# Autodesk Inventor assembly: Frame
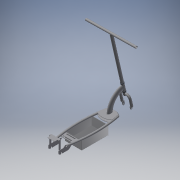
[picture p0: Inventor's stored thumbnail of the model, 180x180]
Saved by Autodesk Inventor 2018 (Build 220112000, 112)
## iProperties
Created: 2018-08-10
Part Number: Frame
Document SubType Name: Assembly
Designer: ruben
Author: ruben
## Documents named in this file (11)
- C:\Users\ruben\Documents\Inventor\Electric-Scooter\Frame\Frame.iam
- C:\Users\ruben\Documents\Inventor\Electric-Scooter\Frame\Rear Wheel Holder.ipt
- C:\Users\ruben\Documents\Inventor\Electric-Scooter\Frame\Footboard - feet protect holder.ipt
- C:\Users\ruben\Documents\Inventor\Electric-Scooter\Frame\Batterybox 2\Batterybox 2.ipt
- C:\Users\ruben\Documents\Inventor\Electric-Scooter\Frame\Tubes.ipt
- C:\Users\ruben\Documents\Inventor\Electric-Scooter\Frame\Handle bars\Handle bars holder plates.ipt
- C:\Users\ruben\Documents\Inventor\Electric-Scooter\Frame\Handle bars\Handle bars holder.ipt
- C:\Users\ruben\Documents\Inventor\Electric-Scooter\Frame\Handle bars\Handle bars holder axle.ipt
- C:\Users\ruben\Documents\Inventor\Electric-Scooter\Transmission\Motor holder slider.ipt
- C:\Users\ruben\Documents\Inventor\Electric-Scooter\Frame\Handle bars\Wheel holder on handle bars axle.ipt
- C:\Users\ruben\Documents\Inventor\Electric-Scooter\Frame\Handle bars\Handle bars.ipt
## Components (12 placed, 10 different names)
1. Rear Wheel Holder:1 — Mate:4, Flush:1, Flush:3, Flush:4, Mate:6, Tangent:5
2. Rear Wheel Holder:2 — Mate:5, Flush:3, Flush:4, Flush:5, Tangent:6, Tangent:7
3. Footboard - feet protect holder:1 — Mate:4, Flush:1, Mate:5, Flush:5
4. Batterybox 2:1 — Mate:8, Mate:9, Mate:10
5. Tubes:1 — Mate:6, Mate:8, Mate:9, Mate:10, Tangent:5, Tangent:6, Tangent:7, Tangent:8, Mate:13, Mate:14, Mate:22, Mate:23, Mate:24
6. Handle bars holder plates:1 — Mate:12, Flush:6, Flush:7
7. Handle bars holder plates:2 — Mate:12, Flush:6, Flush:7, Tangent:8, Mate:13, Mate:14, Mate:15, Mate:16, Mate:17
8. Handle bars holder:1 — Mate:15, Mate:16, Mate:17, Mate:19, Mate:20, Mate:21
9. Handle bars holder axle:1 — Mate:19, Mate:20, Mate:21, Insert:1, Insert:2
10. Motor holder slider:1 — Mate:22, Mate:23, Mate:24
11. Wheel holder on handle bars axle:1 — Insert:1
12. Handle bars:1 — Insert:2
## Relationships (30: Mate 18, Flush 6, Tangent 4, Insert 2)
- Mate:4: Rear Wheel Holder:1 ↔ Footboard - feet protect holder:1
- Flush:1 (85 mm): Rear Wheel Holder:1 ↔ Footboard - feet protect holder:1
- Mate:5: Rear Wheel Holder:2 ↔ Footboard - feet protect holder:1
- Flush:3: Rear Wheel Holder:1 ↔ Rear Wheel Holder:2
- Flush:4: Rear Wheel Holder:1 ↔ Rear Wheel Holder:2
- Mate:6: Rear Wheel Holder:1 ↔ Tubes:1
- Mate:8: Batterybox 2:1 ↔ Tubes:1
- Mate:9: Batterybox 2:1 ↔ Tubes:1
- Mate:10: Batterybox 2:1 ↔ Tubes:1
- Tangent:5: Rear Wheel Holder:1 ↔ Tubes:1
- Flush:5 (4 mm): Rear Wheel Holder:2 ↔ Footboard - feet protect holder:1
- Tangent:6: Rear Wheel Holder:2 ↔ Tubes:1
- Tangent:7: Rear Wheel Holder:2 ↔ Tubes:1
- Mate:12 (20 mm): Handle bars holder plates:1 ↔ Handle bars holder plates:2
- Flush:6: Handle bars holder plates:1 ↔ Handle bars holder plates:2
- Flush:7: Handle bars holder plates:1 ↔ Handle bars holder plates:2
- Tangent:8: Tubes:1 ↔ Handle bars holder plates:2
- Mate:13: Tubes:1 ↔ Handle bars holder plates:2
- Mate:14: Tubes:1 ↔ Handle bars holder plates:2
- Mate:15: Handle bars holder plates:2 ↔ Handle bars holder:1
- Mate:16: Handle bars holder plates:2 ↔ Handle bars holder:1
- Mate:17: Handle bars holder plates:2 ↔ Handle bars holder:1
- Mate:19: Handle bars holder:1 ↔ Handle bars holder axle:1
- Mate:20: Handle bars holder:1 ↔ Handle bars holder axle:1
- Mate:21 (-5 mm): Handle bars holder:1 ↔ Handle bars holder axle:1
- Mate:22: Tubes:1 ↔ Motor holder slider:1
- Mate:23: Tubes:1 ↔ Motor holder slider:1
- Mate:24: Tubes:1 ↔ Motor holder slider:1
- Insert:1 (-1 mm): Handle bars holder axle:1 ↔ Wheel holder on handle bars axle:1
- Insert:2: Handle bars holder axle:1 ↔ Handle bars:1
